# Autodesk Inventor assembly: StatorAssembly
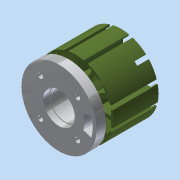
[picture p0: Inventor's stored thumbnail of the model, 180x180]
Saved by Autodesk Inventor 2015 (Build 190159000, 159)
## iProperties
Created: 2015-12-24
Part Number: StatorAssembly
Document SubType Name: Assembly
Designer: Raphael
Author: Raphael
## Documents named in this file (3)
- \\psf\Home\Documents\electric-skateboard\CAD\HubMotor\StatorAssembly.iam
- \\psf\Home\Documents\electric-skateboard\CAD\HubMotor\StatorCore.ipt
- \\psf\Home\Documents\electric-skateboard\CAD\HubMotor\Stator.ipt
## Components (2 placed, 2 different names)
1. StatorCore:1 — Mate:1, Flush:1
2. Stator:1 — Mate:1, Flush:1
## Relationships (2: Mate 1, Flush 1)
- Mate:1: StatorCore:1 ↔ Stator:1
- Flush:1: StatorCore:1 ↔ Stator:1
